# Autodesk Inventor assembly: F_Legs2_MIR
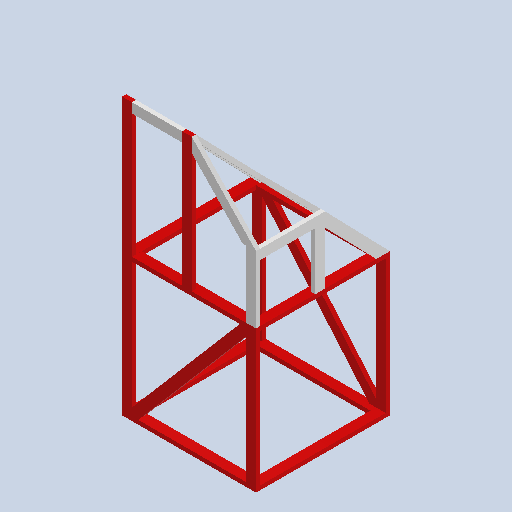
[picture p0: Inventor's stored thumbnail of the model, 512x512]
Saved by Autodesk Inventor 2025 (Build 290162000, 162)
## iProperties
Created: 2024-09-19
Part Number: F_Legs2_MIR
Document SubType Name: Assembly
Designer: localadmin
Author: User
## Documents named in this file (11)
- C:\Users\localadmin\Documents\USCTigerBurn24\Tburn24\F_Legs2\F_Legs2_MIR.iam
- C:\Users\localadmin\Documents\USCTigerBurn24\Tburn24\F_Legs2\8'x2x4_MIR.ipt
- C:\Users\localadmin\Documents\USCTigerBurn24\Tburn24\F_Legs2\3'5x2x4_MIR.ipt
- C:\Users\localadmin\Documents\USCTigerBurn24\Tburn24\F_Legs2\4x2x4_MIR.ipt
- C:\Users\localadmin\Documents\USCTigerBurn24\Tburn24\F_Legs2\44x2x4_MIR.ipt
- C:\Users\localadmin\Documents\USCTigerBurn24\Tburn24\F_Legs2\back_side_MIR.ipt
- C:\Users\localadmin\Documents\USCTigerBurn24\Tburn24\F_Legs2\side-side_MIR.ipt
- C:\Users\localadmin\Documents\USCTigerBurn24\Tburn24\F_Legs2\side-side1_MIR.ipt
- C:\Users\localadmin\Documents\USCTigerBurn24\Tburn24\F_Legs2\side-slant_MIR.ipt
- C:\Users\localadmin\Documents\USCTigerBurn24\Tburn24\F_Legs2\side-side2_MIR.ipt
- C:\Users\localadmin\Documents\USCTigerBurn24\Tburn24\F_Legs2\back-side_MIR.ipt
## Components (23 placed, 10 different names)
1. 8'x2x4_MIR:1 — Flush:3, Flush:2, Flush:1, Flush:5, Flush:4, Flush:14, Flush:13, Flush:8, Flush:12, Flush:10, Mate:3
2. 8'x2x4_MIR:2 — Flush:3, Flush:2, Flush:1, Mate:1, Flush:7, Flush:6, Mate:2, Flush:16, Flush:15, Mate:5, Flush:11, Flush:9
3. 3'5x2x4_MIR:1 — Flush:5, Flush:4
4. 3'5x2x4_MIR:2 — Flush:7, Flush:6, Mate:2, Mate:4
5. 4x2x4_MIR:1 — Flush:14, Flush:13, Flush:8, Flush:29, Flush:20, Flush:17, Mate:7
6. 4x2x4_MIR:2 — Flush:16, Flush:15, Mate:5, Flush:19, Flush:18, Mate:6, Flush:27
7. 4x2x4_MIR:3 — Flush:11, Flush:9, Mate:4
8. 4x2x4_MIR:4 — Flush:12, Flush:10, Mate:3, Flush:28, Mate:13
9. 8'x2x4_MIR:3 — Flush:29, Flush:20, Flush:17, Mate:7, Mate:8, Flush:24, Flush:23, Mate:9, Flush:32
10. 8'x2x4_MIR:4 — Flush:19, Flush:18, Mate:6, Flush:22, Flush:21, Flush:37
11. 3'5x2x4_MIR:3 — Flush:22, Flush:21, Mate:8, Mate:12, Mate:17
12. 3'5x2x4_MIR:4 — Flush:24, Flush:23, Mate:9, Flush:30, Mate:14, Flush:31, Mate:15
13. 44x2x4_MIR:1 — Flush:27
14. 44x2x4_MIR:2 — Flush:28, Mate:13, Mate:12
15. 4x2x4_MIR:5 — Flush:32, Flush:30, Mate:14, Flush:33, Flush:35
16. 4x2x4_MIR:6 — Flush:33, Flush:31, Mate:15, Flush:34, Flush:36, Mate:16, Flush:40
17. back_side_MIR:1 — Flush:34
18. side-side_MIR:1 — Flush:35
19. side-side_MIR:2 — Flush:36, Mate:17, Mate:16, Flush:38
20. side-side1_MIR:1 — Flush:37, Flush:39
21. side-slant_MIR:1 — Flush:38
22. side-side2_MIR:1 — Flush:39
23. back-side_MIR:1 — Flush:40
## Relationships (53: Flush 28, Mate 25)
- Flush:3: 8'x2x4_MIR:1 ↔ 8'x2x4_MIR:2
- Flush:2 (1130.3 mm): 8'x2x4_MIR:1 ↔ 8'x2x4_MIR:2
- Flush:1: 8'x2x4_MIR:1 ↔ 8'x2x4_MIR:2
- Mate:1: 8'x2x4_MIR:2
- Flush:5 [Mate]: 8'x2x4_MIR:1 ↔ 3'5x2x4_MIR:1
- Flush:4 [Mate]: 8'x2x4_MIR:1 ↔ 3'5x2x4_MIR:1
- Flush:7: 8'x2x4_MIR:2 ↔ 3'5x2x4_MIR:2
- Flush:6: 8'x2x4_MIR:2 ↔ 3'5x2x4_MIR:2
- Mate:2: 8'x2x4_MIR:2 ↔ 3'5x2x4_MIR:2
- Flush:14: 8'x2x4_MIR:1 ↔ 4x2x4_MIR:1
- Flush:13: 8'x2x4_MIR:1 ↔ 4x2x4_MIR:1
- Flush:8 [Mate]: 8'x2x4_MIR:1 ↔ 4x2x4_MIR:1
- Flush:16: 8'x2x4_MIR:2 ↔ 4x2x4_MIR:2
- Flush:15: 8'x2x4_MIR:2 ↔ 4x2x4_MIR:2
- Mate:5: 8'x2x4_MIR:2 ↔ 4x2x4_MIR:2
- Flush:11: 8'x2x4_MIR:2 ↔ 4x2x4_MIR:3
- Flush:9: 8'x2x4_MIR:2 ↔ 4x2x4_MIR:3
- Mate:4: 3'5x2x4_MIR:2 ↔ 4x2x4_MIR:3
- Flush:12: 8'x2x4_MIR:1 ↔ 4x2x4_MIR:4
- Flush:10: 8'x2x4_MIR:1 ↔ 4x2x4_MIR:4
- Mate:3: 8'x2x4_MIR:1 ↔ 4x2x4_MIR:4
- Flush:29: 4x2x4_MIR:1 ↔ 8'x2x4_MIR:3
- Flush:20: 4x2x4_MIR:1 ↔ 8'x2x4_MIR:3
- Flush:17: 4x2x4_MIR:1 ↔ 8'x2x4_MIR:3
- Mate:7: 4x2x4_MIR:1 ↔ 8'x2x4_MIR:3
- Flush:19: 4x2x4_MIR:2 ↔ 8'x2x4_MIR:4
- Flush:18: 4x2x4_MIR:2 ↔ 8'x2x4_MIR:4
- Mate:6: 4x2x4_MIR:2 ↔ 8'x2x4_MIR:4
- Flush:22: 8'x2x4_MIR:4 ↔ 3'5x2x4_MIR:3
- Flush:21: 8'x2x4_MIR:4 ↔ 3'5x2x4_MIR:3
- Mate:8: 8'x2x4_MIR:3 ↔ 3'5x2x4_MIR:3
- Flush:24: 8'x2x4_MIR:3 ↔ 3'5x2x4_MIR:4
- Flush:23: 8'x2x4_MIR:3 ↔ 3'5x2x4_MIR:4
- Mate:9: 8'x2x4_MIR:3 ↔ 3'5x2x4_MIR:4
- Flush:27 [Mate]: 4x2x4_MIR:2 ↔ 44x2x4_MIR:1
- Flush:28: 4x2x4_MIR:4 ↔ 44x2x4_MIR:2
- Mate:13: 4x2x4_MIR:4 ↔ 44x2x4_MIR:2
- Mate:12: 3'5x2x4_MIR:3 ↔ 44x2x4_MIR:2
- Flush:32: 8'x2x4_MIR:3 ↔ 4x2x4_MIR:5
- Flush:30: 3'5x2x4_MIR:4 ↔ 4x2x4_MIR:5
- Mate:14: 3'5x2x4_MIR:4 ↔ 4x2x4_MIR:5
- Flush:33 (546.1 mm): 4x2x4_MIR:5 ↔ 4x2x4_MIR:6
- Flush:31: 3'5x2x4_MIR:4 ↔ 4x2x4_MIR:6
- Mate:15: 3'5x2x4_MIR:4 ↔ 4x2x4_MIR:6
- Flush:34 [Mate]: 4x2x4_MIR:6 ↔ back_side_MIR:1
- Flush:35 [Mate]: 4x2x4_MIR:5 ↔ side-side_MIR:1
- Flush:36: 4x2x4_MIR:6 ↔ side-side_MIR:2
- Mate:17: 3'5x2x4_MIR:3 ↔ side-side_MIR:2
- Mate:16: 4x2x4_MIR:6 ↔ side-side_MIR:2
- Flush:37 [Mate]: 8'x2x4_MIR:4 ↔ side-side1_MIR:1
- Flush:38 [Mate]: side-side_MIR:2 ↔ side-slant_MIR:1
- Flush:39 [Mate]: side-side1_MIR:1 ↔ side-side2_MIR:1
- Flush:40 [Mate]: 4x2x4_MIR:6 ↔ back-side_MIR:1
